# Autodesk Inventor assembly: a shock absorber
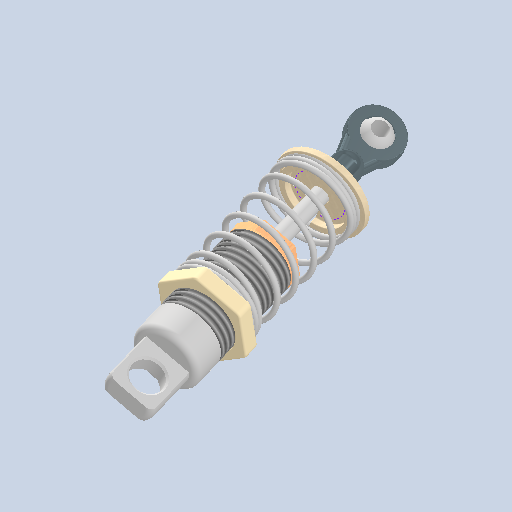
[picture p0: Inventor's stored thumbnail of the model, 512x512]
Saved by Autodesk Inventor 2024 (Build 280153000, 153)
## iProperties
Created: 2023-07-07
Part Number: a shock absorber
Document SubType Name: Assembly
Designer: birud
Author: birud
## Documents named in this file (5)
- C:\Users\_Astitva_Aryan_\Downloads\ES101_Components_Group5\Components_derived\a shock absorber.iam
- C:\Users\_Astitva_Aryan_\Downloads\ES101_Components_Group5\Components_derived\SA Shock Spring Adjustment Nut.ipt
- C:\Users\_Astitva_Aryan_\Downloads\ES101_Components_Group5\Components_derived\SA Suspension Spring.ipt
- C:\Users\_Astitva_Aryan_\Downloads\ES101_Components_Group5\Components_derived\a shock body.iam
- C:\Users\_Astitva_Aryan_\Downloads\ES101_Components_Group5\Components_derived\a shock strut.iam
## Components (4 placed, 4 different names)
1. SA Shock Spring Adjustment Nut:1 — Mate:1, Mate:2, Flush:1, Angle:1, Mate:5, Angle:2
2. SA Suspension Spring:1 — Mate:1, Mate:4, Mate:5
3. a shock body:1 [sub-assembly] — Mate:2, Flush:1, Angle:1, Mate:3
4. a shock strut:1 [sub-assembly] — Mate:3, Mate:4, Angle:2
## Relationships (8: Mate 5, Angle 2, Flush 1)
- Mate:1: SA Shock Spring Adjustment Nut:1 ↔ SA Suspension Spring:1
- Mate:2: SA Shock Spring Adjustment Nut:1 ↔ a shock body:1
- Flush:1 (-101.6762 mm): SA Shock Spring Adjustment Nut:1 ↔ a shock body:1
- Angle:1 (0 deg): SA Shock Spring Adjustment Nut:1 ↔ a shock body:1
- Mate:3: a shock body:1 ↔ a shock strut:1
- Mate:4: SA Suspension Spring:1 ↔ a shock strut:1
- Mate:5: SA Shock Spring Adjustment Nut:1 ↔ SA Suspension Spring:1
- Angle:2 (0 deg): SA Shock Spring Adjustment Nut:1 ↔ a shock strut:1
